# Autodesk Inventor assembly: Chuck - V2
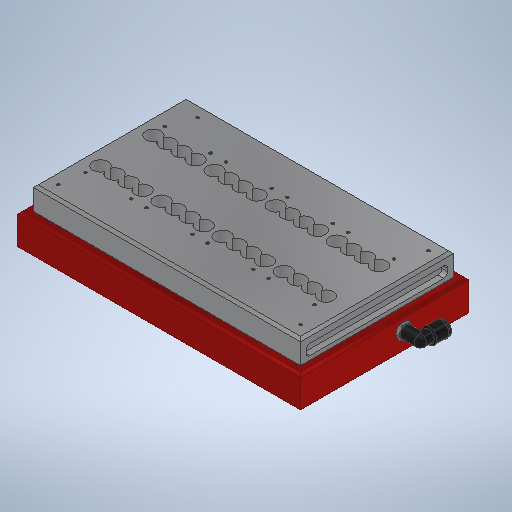
[picture p0: Inventor's stored thumbnail of the model, 512x512]
Saved by Autodesk Inventor 2025 (Build 290162000, 162)
## iProperties
Created: 2021-03-04
Part Number: Chuck - V2
Document SubType Name: Assembly
Designer: caleb
Author: caleb
## Documents named in this file (5)
- C:\Users\cfang\Desktop\nebraska-silicon-lab\Hardware\ETL\Module Assembly\Chuck - V3\Chuck - V3.iam
- C:\Users\cfang\Desktop\nebraska-silicon-lab\Hardware\ETL\Module Assembly\Chuck - V3\Chuck - V3.ipt
- C:\Users\cfang\Desktop\nebraska-silicon-lab\Hardware\ETL\Module Assembly\Chuck - V3\5486K121_Weld-Spatter-Resistant Push-to-Connect Tube Fitting\5486K121_Weld-Spatter-Resistant Push-to-Connect Tube Fitting.ipt
- C:\Users\cfang\Desktop\nebraska-silicon-lab\Hardware\ETL\Module Assembly\Tamale Assembly Plate V6a\Tamale Assembly Plate V6a.ipt
- C:\Users\cfang\Desktop\nebraska-silicon-lab\Hardware\ETL\Module Assembly\Chuck - V3\93600A304_316 Stainless Steel Dowel Pin\93600A304_316 Stainless Steel Dowel Pin.ipt
## Components (7 placed, 4 different names)
1. Chuck - V3:1 — Insert:6, Mate:1, Angle:1, Insert:7, Insert:8, Insert:9, Insert:10
2. 5486K121_Weld-Spatter-Resistant Push-to-Connect Tube Fitting:1 — Insert:6
3. Tamale Assembly Plate V6a:1 — Mate:1, Angle:1, Tangent:1, Tangent:2
4. 93600A304_316 Stainless Steel Dowel Pin:1 — Insert:7
5. 93600A304_316 Stainless Steel Dowel Pin:2 — Insert:8, Tangent:2
6. 93600A304_316 Stainless Steel Dowel Pin:3 — Insert:10
7. 93600A304_316 Stainless Steel Dowel Pin:4 — Insert:9, Tangent:1
## Relationships (9: Insert 5, Tangent 2, Mate 1, Angle 1)
- Insert:6: Chuck - V3:1 ↔ 5486K121_Weld-Spatter-Resistant Push-to-Connect Tube Fitting:1
- Mate:1: Chuck - V3:1 ↔ Tamale Assembly Plate V6a:1
- Angle:1 (0 deg): Chuck - V3:1 ↔ Tamale Assembly Plate V6a:1
- Insert:7 (-5 mm): Chuck - V3:1 ↔ 93600A304_316 Stainless Steel Dowel Pin:1
- Insert:8 (-5 mm): Chuck - V3:1 ↔ 93600A304_316 Stainless Steel Dowel Pin:2
- Insert:9 (-5 mm): Chuck - V3:1 ↔ 93600A304_316 Stainless Steel Dowel Pin:4
- Insert:10 (-5 mm): Chuck - V3:1 ↔ 93600A304_316 Stainless Steel Dowel Pin:3
- Tangent:1: Tamale Assembly Plate V6a:1 ↔ 93600A304_316 Stainless Steel Dowel Pin:4
- Tangent:2: Tamale Assembly Plate V6a:1 ↔ 93600A304_316 Stainless Steel Dowel Pin:2
